# Autodesk Inventor assembly: R-Upright20181
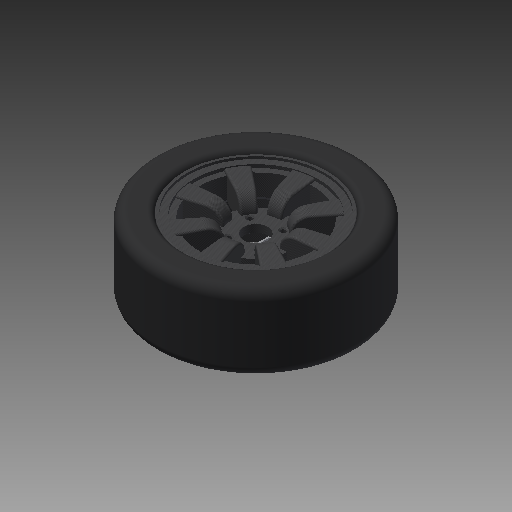
[picture p0: Inventor's stored thumbnail of the model, 512x512]
Saved by Autodesk Inventor 2018.2 (Build 222227000, 227)
## iProperties
Created: 2018-05-19
Part Number: R-Upright20181
Material: 一般
Document SubType Name: Assembly
Designer: ku_sk
Title: D:\ku_sk\ドキュメント\Inventor\Aero\KS-15\全体アッセンブリ解析用モデル\body\sus\R-Upright2018.stp
Author: ku_sk
Sending System: Autodesk Inventor 2018
Preprocessor: ST-DEVELOPER v17
## Documents named in this file (5)
- D:\ku_sk\ドキュメント\Inventor\Aero\KS-15\全体アッセンブリ解析用モデル\body\sus\R-Upright20181.iam
- D:\ku_sk\ドキュメント\Inventor\Aero\KS-15\全体アッセンブリ解析用モデル\body\sus\Rear Upright 4.161.ipt
- D:\ku_sk\ドキュメント\Inventor\Aero\KS-15\全体アッセンブリ解析用モデル\body\sus\R-Upright Bracket 20181.ipt
- D:\ku_sk\ドキュメント\Inventor\Aero\KS-15\全体アッセンブリ解析用モデル\body\sus\R-Sim13 20181.ipt
- D:\ku_sk\ドキュメント\Inventor\Aero\KS-15\全体アッセンブリ解析用モデル\body\sus\2015Wheel watanabe1.ipt
## Components (4 placed, 4 different names)
1. Rear Upright 4.161:1 — メイト:2, メイト:1
2. R-Upright Bracket 20181:1
3. R-Sim13 20181:1
4. 2015Wheel watanabe1:1 — メイト:2, メイト:1
## Relationships (2: Mate 2)
- メイト:2 [Mate] (49 mm): Rear Upright 4.161:1 ↔ 2015Wheel watanabe1:1
- メイト:1 [Mate]: Rear Upright 4.161:1 ↔ 2015Wheel watanabe1:1
